# Autodesk Inventor assembly: 1590E
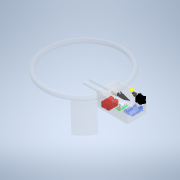
[picture p0: Inventor's stored thumbnail of the model, 180x180]
Saved by Autodesk Inventor 2021 (Build 250183000, 183)
## iProperties
Created: 2015-07-13
Part Number: 1590E
Document SubType Name: Assembly
Designer: elmar
Sending System: Autodesk Inventor 2015
Preprocessor: ST-DEVELOPER v15.6
Title: E:\Eng\Customer Service\Drawings\1590\STEP\1590E.stp
Author: mbeerman
## Documents named in this file (11)
- C:\Users\Eric\OneDrive\Inventor\LEGEND\PressureBuildingHeaterController\1590E.iam
- C:\Users\Eric\OneDrive\Inventor\LEGEND\PressureBuildingHeaterController\1590E BOX.ipt
- C:\Users\Eric\OneDrive\Inventor\LEGEND\PressureBuildingHeaterController\1590D-DD-E LID.ipt
- C:\Users\Eric\OneDrive\Inventor\LEGEND\PressureBuildingHeaterController\SC530 (screw #6-32X 1_2'' FH).ipt
- C:\Users\Eric\OneDrive\Inventor\LEGEND\PressureBuildingHeaterController\701wx202.iam
- C:\Users\Eric\OneDrive\Inventor\LEGEND\PressureBuildingHeaterController\G3NA_220B.ipt
- C:\Users\Eric\OneDrive\Inventor\LEGEND\PressureBuildingHeaterController\arduino uno.ipt
- C:\Users\Eric\OneDrive\Inventor\LEGEND\PressureBuildingHeaterController\DewarObstructions.ipt
- C:\Users\Eric\OneDrive\Inventor\LEGEND\PressureBuildingHeaterController\RA1113112R.ipt
- C:\Users\Eric\OneDrive\Inventor\LEGEND\PressureBuildingHeaterController\CFM12S-1060321.ipt
- C:\Users\Eric\OneDrive\Inventor\LEGEND\PressureBuildingHeaterController\Pressure transducer with connector.iam
## Components (15 placed, 10 different names)
1. 1590E BOX:1 — Mate:6, Mate:14, Mate:15, Mate:16, Mate:17, Angle:1, Mate:18, Mate:19, Mate:20, Mate:21, Mate:23, Insert:1, Mate:24, Mate:25, Mate:26
2. 1590D-DD-E LID:1
3. SC530 (screw #6-32X 1_2'' FH):5
4. SC530 (screw #6-32X 1_2'' FH):6
5. SC530 (screw #6-32X 1_2'' FH):1
6. SC530 (screw #6-32X 1_2'' FH):2
7. SC530 (screw #6-32X 1_2'' FH):3
8. SC530 (screw #6-32X 1_2'' FH):4
9. 701wx202:1 [sub-assembly] — Angle:1, Mate:18, Mate:21
10. G3NA_220B:1 — Mate:17, Mate:24, Mate:25
11. arduino uno:1 — Mate:6, Mate:23, Mate:27
12. DewarObstructions:1 — Mate:14, Mate:15, Mate:16
13. RA1113112R:1 — Mate:19, Mate:20
14. CFM12S-1060321:2 — Mate:26, Mate:27
15. Pressure transducer with connector:1 [sub-assembly] — Insert:1
## Relationships (16: Mate 14, Angle 1, Insert 1)
- Mate:6 (10 mm): 1590E BOX:1 ↔ arduino uno:1
- Mate:14: 1590E BOX:1 ↔ DewarObstructions:1
- Mate:15 (30 mm): 1590E BOX:1 ↔ DewarObstructions:1
- Mate:16 (70 mm): 1590E BOX:1 ↔ DewarObstructions:1
- Mate:17 (0.5 mm): 1590E BOX:1 ↔ G3NA_220B:1
- Angle:1 (0 deg): 1590E BOX:1 ↔ 701wx202:1
- Mate:18: 1590E BOX:1 ↔ 701wx202:1
- Mate:19 (10 mm): 1590E BOX:1 ↔ RA1113112R:1
- Mate:20 (1 mm): 1590E BOX:1 ↔ RA1113112R:1
- Mate:21 (10 mm): 1590E BOX:1 ↔ 701wx202:1
- Mate:23: 1590E BOX:1 ↔ arduino uno:1
- Insert:1 (10 mm): 1590E BOX:1 ↔ Pressure transducer with connector:1
- Mate:24 (10 mm): 1590E BOX:1 ↔ G3NA_220B:1
- Mate:25 (15 mm): 1590E BOX:1 ↔ G3NA_220B:1
- Mate:26 (10 mm): 1590E BOX:1 ↔ CFM12S-1060321:2
- Mate:27 (15 mm): arduino uno:1 ↔ CFM12S-1060321:2
